# Autodesk Inventor assembly: V0_PLENUM_1515_Extrusion_V6
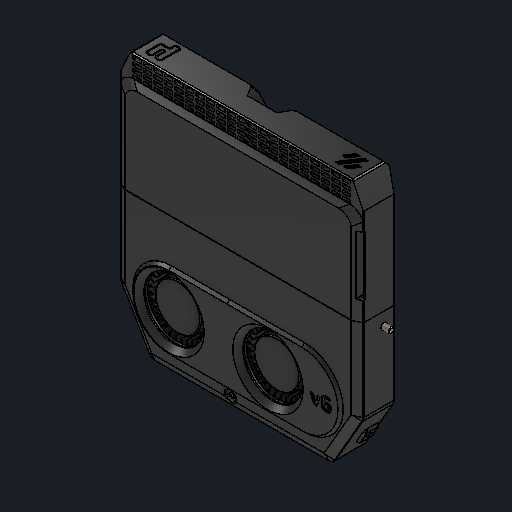
[picture p0: Inventor's stored thumbnail of the model, 512x512]
Saved by Autodesk Inventor 2026.2 (Build 302298000, 298)
## iProperties
Created: 2025-11-15
Part Number: V0_PLENUM_1515_Extrusion_V6
Document SubType Name: Assembly
Designer: JoshuaEah
Sending System: Autodesk Translation Framework v14.21.0.0
Preprocessor: ST-DEVELOPER v20.1
Title: V0_PLENUM_1515_Extrusion_V6.step
## Documents named in this file (12)
- C:\Users\JoshuaEah\Documents\GitHub\Voron-0\CAD\Extras\Nevermore V6 Micro\Nevermore V6 Micro.iam
- C:\Users\JoshuaEah\Documents\GitHub\Voron-0\CAD\Extras\Nevermore V6 Micro\Fan_Clamps.ipt
- C:\Users\JoshuaEah\Documents\GitHub\Voron-0\CAD\Extras\Nevermore V6 Micro\Plenum_Lid.ipt
- C:\Users\JoshuaEah\Documents\GitHub\Voron-0\CAD\Extras\Nevermore V6 Micro\Plenum.ipt
- C:\Users\JoshuaEah\Documents\GitHub\Voron-0\CAD\Extras\Nevermore V6 Micro\Wago_221.ipt
- C:\Users\JoshuaEah\Documents\GitHub\Voron-0\CAD\Extras\Nevermore V6 Micro\Wire_connector.ipt
- C:\Users\JoshuaEah\Documents\GitHub\Voron-0\CAD\Hardware\Electronics\Parts\5015 Fan.iam
- C:\Users\JoshuaEah\Documents\GitHub\Voron-0\CAD\Hardware\Fasteners\M3 Threaded Insert.ipt
- C:\Users\JoshuaEah\Documents\GitHub\Voron-0\CAD\Hardware\Fasteners\M3x16 BHCS.ipt
- C:\Users\JoshuaEah\Documents\GitHub\Voron-0\CAD\Hardware\Fasteners\M3x20 SHCS.ipt
- C:\Users\JoshuaEah\Documents\GitHub\Voron-0\CAD\Hardware\Fasteners\M3x8 BHCS.ipt
- C:\Users\JoshuaEah\Documents\GitHub\Voron-0\CAD\Extras\Nevermore V6 Micro\V6 Micro Cartridge.ipt
## Components (14 placed, 11 different names)
1. Plenum:1 — Insert:1, Insert:2, Insert:3, Insert:4, Angle:1, Insert:7, Insert:8, Angle:2, Insert:9, Insert:10
2. Plenum_Lid:1 — Insert:5, Insert:6
3. Fan_Clamps:1
4. Wago_221:1
5. Wire_connector:1
6. M3x16 BHCS:1 — Insert:2
7. M3 Threaded Insert:1 — Insert:1
8. M3x20 SHCS:1 — Insert:3
9. M3x16 BHCS:2 — Insert:4
10. M3x8 BHCS:1 — Insert:5
11. M3 Threaded Insert:2 — Insert:6
12. 5015 Fan:1 [sub-assembly] — Angle:1, Insert:7
13. 5015 Fan:2 [sub-assembly] — Insert:8, Angle:2
14. V6 Micro Cartridge:1 — Insert:9, Insert:10
## Relationships (12: Insert 10, Angle 2)
- Insert:1: Plenum:1 ↔ M3 Threaded Insert:1
- Insert:2: Plenum:1 ↔ M3x16 BHCS:1
- Insert:3: Plenum:1 ↔ M3x20 SHCS:1
- Insert:4: Plenum:1 ↔ M3x16 BHCS:2
- Insert:5: Plenum_Lid:1 ↔ M3x8 BHCS:1
- Insert:6: Plenum_Lid:1 ↔ M3 Threaded Insert:2
- Angle:1 (0 deg): Plenum:1 ↔ 5015 Fan:1
- Insert:7: Plenum:1 ↔ 5015 Fan:1
- Insert:8: Plenum:1 ↔ 5015 Fan:2
- Angle:2 (0 deg): Plenum:1 ↔ 5015 Fan:2
- Insert:9: Plenum:1 ↔ V6 Micro Cartridge:1
- Insert:10: Plenum:1 ↔ V6 Micro Cartridge:1
